# Autodesk Inventor assembly: CCM_Unit
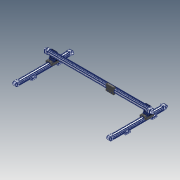
[picture p0: Inventor's stored thumbnail of the model, 180x180]
Saved by Autodesk Inventor 2020 (Build 240168000, 168)
## iProperties
Created: 2021-02-24
Part Number: CCM_Unit
Document SubType Name: Assembly
Designer: magnarecta
Author: magnarecta
## Documents named in this file (5)
- C:\Users\lvglv\Documents\GitHub\Eto_Project\Hardware\Asem\CCM_Unit.iam
- C:\Users\lvglv\Documents\GitHub\Eto_Project\Hardware\Parts\CCM\CCM motion linear guide rail\CCM_UNIT\CCM_Unit_C.iam
- C:\Users\lvglv\Documents\GitHub\Eto_Project\Hardware\Parts\CCM\CCM motion linear guide rail\CCM_UNIT\CCM_Unit_A.iam
- C:\Users\lvglv\Documents\GitHub\Eto_Project\Hardware\Parts\CCM\CCM motion linear guide rail\CCM_UNIT\CCM_Unit_B.iam
- C:\Users\lvglv\Documents\GitHub\Eto_Project\Hardware\Parts\CCM\CCM motion linear guide rail\CCM_UNIT\Ly1__1.ipt
## Components (5 placed, 4 different names)
1. CCM_Unit_C:1 [sub-assembly] — メイト:6, 角度:1, フラッシュ:5, フラッシュ:6, メイト:7, フラッシュ:7
2. CCM_Unit_A:1 [sub-assembly] — フラッシュ:1, フラッシュ:2, フラッシュ:3, フラッシュ:4, メイト:1, メイト:2, メイト:8
3. CCM_Unit_B:1 [sub-assembly] — フラッシュ:1, フラッシュ:2, フラッシュ:3, フラッシュ:4, メイト:3, メイト:4, メイト:5
4. Ly1__1:1 — メイト:1, メイト:2, メイト:6, 角度:1, フラッシュ:5, フラッシュ:7, メイト:8
5. Ly1__1:2 — メイト:3, メイト:4, メイト:5, フラッシュ:6, メイト:7
## Relationships (16: Mate 8, Flush 7, Angle 1)
- フラッシュ:1 [Flush]: CCM_Unit_A:1 ↔ CCM_Unit_B:1
- フラッシュ:2 [Flush]: CCM_Unit_A:1 ↔ CCM_Unit_B:1
- フラッシュ:3 [Flush]: CCM_Unit_A:1 ↔ CCM_Unit_B:1
- フラッシュ:4 [Flush]: CCM_Unit_A:1 ↔ CCM_Unit_B:1
- メイト:1 [Mate]: CCM_Unit_A:1 ↔ Ly1__1:1
- メイト:2 [Mate]: CCM_Unit_A:1 ↔ Ly1__1:1
- メイト:3 [Mate]: CCM_Unit_B:1 ↔ Ly1__1:2
- メイト:4 [Mate]: CCM_Unit_B:1 ↔ Ly1__1:2
- メイト:5 [Mate]: CCM_Unit_B:1 ↔ Ly1__1:2
- メイト:6 [Mate]: CCM_Unit_C:1 ↔ Ly1__1:1
- 角度:1 [Angle] (0 deg): CCM_Unit_C:1 ↔ Ly1__1:1
- フラッシュ:5 [Flush]: CCM_Unit_C:1 ↔ Ly1__1:1
- フラッシュ:6 [Flush]: CCM_Unit_C:1 ↔ Ly1__1:2
- メイト:7 [Mate]: CCM_Unit_C:1 ↔ Ly1__1:2
- フラッシュ:7 [Flush] (0.5 mm): CCM_Unit_C:1 ↔ Ly1__1:1
- メイト:8 [Mate]: CCM_Unit_A:1 ↔ Ly1__1:1
